# Autodesk Inventor assembly: Custom Lift
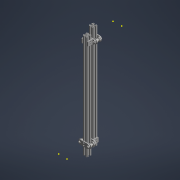
[picture p0: Inventor's stored thumbnail of the model, 180x180]
Saved by Autodesk Inventor 2022 (Build 260153000, 153)
## iProperties
Part Number: Custom Lift
Document SubType Name: Assembly
Designer: izack
Author: izack
## Documents named in this file (7)
- D:\Robotics\ComputerAidedDesign\2021-22\FTC\#12456 Big Red\Verical lift\Custom Lift\Custom Lift.iam
- D:\Robotics\ComputerAidedDesign\2021-22\FTC\#12456 Big Red\Verical lift\Custom Lift\15mm Extrusion - 420mm - 90° Ends.ipt
- D:\Robotics\ComputerAidedDesign\2021-22\FTC\#12456 Big Red\Verical lift\Custom Lift\8mm x 12mm x 3.5mm Flanged Bearing - 10 Pack.ipt
- D:\Robotics\ComputerAidedDesign\2021-22\FTC\#12456 Big Red\Verical lift\Custom Lift\Stationary Bracket.ipt
- D:\Robotics\ComputerAidedDesign\2021-22\FTC\#12456 Big Red\Verical lift\Custom Lift\5mm Hex to 8mm Round Bearing Insert - 20 Pack.ipt
- D:\Robotics\ComputerAidedDesign\2021-22\FTC\#12456 Big Red\Verical lift\Custom Lift\Stationary bracket aligner.ipt
- D:\Robotics\ComputerAidedDesign\2021-22\FTC\#12456 Big Red\Verical lift\Custom Lift\5mm x 90mm Hex Shaft - 4 Pack.ipt
## Components (26 placed, 6 different names)
1. 15mm Extrusion - 420mm - 90° Ends:1 — Mate:2, Flush:1, Tangent:1, Tangent:2, Tangent:3, Tangent:4, Tangent:5, Tangent:6, Tangent:7, Mate:16, Mate:21, Mate:22, Flush:12
2. 8mm x 12mm x 3.5mm Flanged Bearing - 10 Pack:1 — Mate:13, Mate:14, Tangent:6, Tangent:7
3. 8mm x 12mm x 3.5mm Flanged Bearing - 10 Pack:2 — Mate:12, Mate:15, Tangent:4, Tangent:5
4. 8mm x 12mm x 3.5mm Flanged Bearing - 10 Pack:3 — Mate:5, Tangent:3, Mate:8, Mate:9
5. 8mm x 12mm x 3.5mm Flanged Bearing - 10 Pack:4 — Mate:5, Tangent:1, Tangent:2, Mate:10, Mate:11
6. 15mm Extrusion - 420mm - 90° Ends:2 — Mate:2, Flush:1, Mate:6, Mate:7, Flush:11, Tangent:8, Tangent:9, Tangent:10, Tangent:11, Tangent:12, Tangent:13, Tangent:14, Tangent:15, Mate:31
7. Stationary Bracket:1 — Mate:6, Mate:7, Flush:3, Flush:6, Flush:7, Flush:8, Mate:18, Flush:11
8. 5mm Hex to 8mm Round Bearing Insert - 20 Pack:1 — Mate:10, Mate:11, Flush:4, Mate:20
9. 5mm Hex to 8mm Round Bearing Insert - 20 Pack:2 — Mate:8, Mate:9, Flush:3, Flush:4, Mate:19
10. 5mm Hex to 8mm Round Bearing Insert - 20 Pack:3 — Mate:12, Mate:15, Flush:5, Mate:17
11. 5mm Hex to 8mm Round Bearing Insert - 20 Pack:4 — Mate:13, Mate:14, Flush:5, Flush:6
12. Stationary bracket aligner:1 — Mate:16, Flush:7, Flush:8, Flush:9, Flush:10
13. 5mm x 90mm Hex Shaft - 4 Pack:1 — Mate:19, Mate:20, Flush:9
14. 5mm x 90mm Hex Shaft - 4 Pack:2 — Mate:17, Mate:18, Flush:10
15. Stationary Bracket:2 — Mate:21, Mate:22, Flush:12, Flush:15, Flush:16, Flush:17, Mate:32
16. 8mm x 12mm x 3.5mm Flanged Bearing - 10 Pack:5 — Tangent:9, Tangent:14, Mate:23, Mate:29
17. 8mm x 12mm x 3.5mm Flanged Bearing - 10 Pack:6 — Tangent:10, Tangent:15, Mate:25, Mate:28
18. 8mm x 12mm x 3.5mm Flanged Bearing - 10 Pack:7 — Tangent:11, Tangent:12, Mate:26, Mate:27
19. 8mm x 12mm x 3.5mm Flanged Bearing - 10 Pack:8 — Tangent:8, Tangent:13, Mate:24, Mate:30
20. 5mm Hex to 8mm Round Bearing Insert - 20 Pack:5 — Mate:23, Mate:29, Flush:14, Flush:15
21. 5mm Hex to 8mm Round Bearing Insert - 20 Pack:6 — Mate:24, Mate:30, Flush:13, Flush:16
22. 5mm Hex to 8mm Round Bearing Insert - 20 Pack:7 — Mate:25, Mate:28, Flush:14
23. 5mm Hex to 8mm Round Bearing Insert - 20 Pack:8 — Mate:26, Mate:27, Flush:13
24. Stationary bracket aligner:2 — Mate:31, Flush:17, Mate:32, Mate:33, Mate:34, Mate:35, Mate:36, Flush:18, Flush:19
25. 5mm x 90mm Hex Shaft - 4 Pack:3 — Mate:34, Mate:35, Flush:19
26. 5mm x 90mm Hex Shaft - 4 Pack:4 — Mate:33, Mate:36, Flush:18
## Relationships (66: Mate 33, Flush 18, Tangent 15)
- Mate:2 (4 mm): 15mm Extrusion - 420mm - 90° Ends:1 ↔ 15mm Extrusion - 420mm - 90° Ends:2
- Flush:1: 15mm Extrusion - 420mm - 90° Ends:1 ↔ 15mm Extrusion - 420mm - 90° Ends:2
- Mate:5: 8mm x 12mm x 3.5mm Flanged Bearing - 10 Pack:3 ↔ 8mm x 12mm x 3.5mm Flanged Bearing - 10 Pack:4
- Tangent:1: 15mm Extrusion - 420mm - 90° Ends:1 ↔ 8mm x 12mm x 3.5mm Flanged Bearing - 10 Pack:4
- Tangent:2: 15mm Extrusion - 420mm - 90° Ends:1 ↔ 8mm x 12mm x 3.5mm Flanged Bearing - 10 Pack:4
- Tangent:3: 15mm Extrusion - 420mm - 90° Ends:1 ↔ 8mm x 12mm x 3.5mm Flanged Bearing - 10 Pack:3
- Mate:6: 15mm Extrusion - 420mm - 90° Ends:2 ↔ Stationary Bracket:1
- Mate:7: 15mm Extrusion - 420mm - 90° Ends:2 ↔ Stationary Bracket:1
- Mate:8: 8mm x 12mm x 3.5mm Flanged Bearing - 10 Pack:3 ↔ 5mm Hex to 8mm Round Bearing Insert - 20 Pack:2
- Mate:9: 8mm x 12mm x 3.5mm Flanged Bearing - 10 Pack:3 ↔ 5mm Hex to 8mm Round Bearing Insert - 20 Pack:2
- Flush:3: Stationary Bracket:1 ↔ 5mm Hex to 8mm Round Bearing Insert - 20 Pack:2
- Mate:10: 8mm x 12mm x 3.5mm Flanged Bearing - 10 Pack:4 ↔ 5mm Hex to 8mm Round Bearing Insert - 20 Pack:1
- Mate:11: 8mm x 12mm x 3.5mm Flanged Bearing - 10 Pack:4 ↔ 5mm Hex to 8mm Round Bearing Insert - 20 Pack:1
- Flush:4: 5mm Hex to 8mm Round Bearing Insert - 20 Pack:1 ↔ 5mm Hex to 8mm Round Bearing Insert - 20 Pack:2
- Mate:12: 8mm x 12mm x 3.5mm Flanged Bearing - 10 Pack:2 ↔ 5mm Hex to 8mm Round Bearing Insert - 20 Pack:3
- Mate:13: 8mm x 12mm x 3.5mm Flanged Bearing - 10 Pack:1 ↔ 5mm Hex to 8mm Round Bearing Insert - 20 Pack:4
- Mate:14: 8mm x 12mm x 3.5mm Flanged Bearing - 10 Pack:1 ↔ 5mm Hex to 8mm Round Bearing Insert - 20 Pack:4
- Mate:15: 8mm x 12mm x 3.5mm Flanged Bearing - 10 Pack:2 ↔ 5mm Hex to 8mm Round Bearing Insert - 20 Pack:3
- Tangent:4: 15mm Extrusion - 420mm - 90° Ends:1 ↔ 8mm x 12mm x 3.5mm Flanged Bearing - 10 Pack:2
- Tangent:5: 15mm Extrusion - 420mm - 90° Ends:1 ↔ 8mm x 12mm x 3.5mm Flanged Bearing - 10 Pack:2
- Tangent:6: 15mm Extrusion - 420mm - 90° Ends:1 ↔ 8mm x 12mm x 3.5mm Flanged Bearing - 10 Pack:1
- Tangent:7: 15mm Extrusion - 420mm - 90° Ends:1 ↔ 8mm x 12mm x 3.5mm Flanged Bearing - 10 Pack:1
- Flush:5: 5mm Hex to 8mm Round Bearing Insert - 20 Pack:3 ↔ 5mm Hex to 8mm Round Bearing Insert - 20 Pack:4
- Flush:6: Stationary Bracket:1 ↔ 5mm Hex to 8mm Round Bearing Insert - 20 Pack:4
- Mate:16: 15mm Extrusion - 420mm - 90° Ends:1 ↔ Stationary bracket aligner:1
- Flush:7: Stationary Bracket:1 ↔ Stationary bracket aligner:1
- Flush:8: Stationary Bracket:1 ↔ Stationary bracket aligner:1
- Mate:17: 5mm Hex to 8mm Round Bearing Insert - 20 Pack:3 ↔ 5mm x 90mm Hex Shaft - 4 Pack:2
- Mate:18: Stationary Bracket:1 ↔ 5mm x 90mm Hex Shaft - 4 Pack:2
- Mate:19: 5mm Hex to 8mm Round Bearing Insert - 20 Pack:2 ↔ 5mm x 90mm Hex Shaft - 4 Pack:1
- Mate:20: 5mm Hex to 8mm Round Bearing Insert - 20 Pack:1 ↔ 5mm x 90mm Hex Shaft - 4 Pack:1
- Flush:9 (-2 mm): Stationary bracket aligner:1 ↔ 5mm x 90mm Hex Shaft - 4 Pack:1
- Flush:10 (-2 mm): Stationary bracket aligner:1 ↔ 5mm x 90mm Hex Shaft - 4 Pack:2
- Flush:11 (10 mm): 15mm Extrusion - 420mm - 90° Ends:2 ↔ Stationary Bracket:1
- Mate:21: 15mm Extrusion - 420mm - 90° Ends:1 ↔ Stationary Bracket:2
- Mate:22: 15mm Extrusion - 420mm - 90° Ends:1 ↔ Stationary Bracket:2
- Flush:12 (10 mm): 15mm Extrusion - 420mm - 90° Ends:1 ↔ Stationary Bracket:2
- Tangent:8: 15mm Extrusion - 420mm - 90° Ends:2 ↔ 8mm x 12mm x 3.5mm Flanged Bearing - 10 Pack:8
- Tangent:9: 15mm Extrusion - 420mm - 90° Ends:2 ↔ 8mm x 12mm x 3.5mm Flanged Bearing - 10 Pack:5
- Tangent:10: 15mm Extrusion - 420mm - 90° Ends:2 ↔ 8mm x 12mm x 3.5mm Flanged Bearing - 10 Pack:6
- Tangent:11: 15mm Extrusion - 420mm - 90° Ends:2 ↔ 8mm x 12mm x 3.5mm Flanged Bearing - 10 Pack:7
- Tangent:12: 15mm Extrusion - 420mm - 90° Ends:2 ↔ 8mm x 12mm x 3.5mm Flanged Bearing - 10 Pack:7
- Tangent:13: 15mm Extrusion - 420mm - 90° Ends:2 ↔ 8mm x 12mm x 3.5mm Flanged Bearing - 10 Pack:8
- Tangent:14: 15mm Extrusion - 420mm - 90° Ends:2 ↔ 8mm x 12mm x 3.5mm Flanged Bearing - 10 Pack:5
- Tangent:15: 15mm Extrusion - 420mm - 90° Ends:2 ↔ 8mm x 12mm x 3.5mm Flanged Bearing - 10 Pack:6
- Mate:23: 8mm x 12mm x 3.5mm Flanged Bearing - 10 Pack:5 ↔ 5mm Hex to 8mm Round Bearing Insert - 20 Pack:5
- Mate:24: 8mm x 12mm x 3.5mm Flanged Bearing - 10 Pack:8 ↔ 5mm Hex to 8mm Round Bearing Insert - 20 Pack:6
- Mate:25: 8mm x 12mm x 3.5mm Flanged Bearing - 10 Pack:6 ↔ 5mm Hex to 8mm Round Bearing Insert - 20 Pack:7
- Mate:26: 8mm x 12mm x 3.5mm Flanged Bearing - 10 Pack:7 ↔ 5mm Hex to 8mm Round Bearing Insert - 20 Pack:8
- Mate:27: 8mm x 12mm x 3.5mm Flanged Bearing - 10 Pack:7 ↔ 5mm Hex to 8mm Round Bearing Insert - 20 Pack:8
- Mate:28: 8mm x 12mm x 3.5mm Flanged Bearing - 10 Pack:6 ↔ 5mm Hex to 8mm Round Bearing Insert - 20 Pack:7
- Mate:29: 8mm x 12mm x 3.5mm Flanged Bearing - 10 Pack:5 ↔ 5mm Hex to 8mm Round Bearing Insert - 20 Pack:5
- Mate:30: 8mm x 12mm x 3.5mm Flanged Bearing - 10 Pack:8 ↔ 5mm Hex to 8mm Round Bearing Insert - 20 Pack:6
- Flush:13: 5mm Hex to 8mm Round Bearing Insert - 20 Pack:6 ↔ 5mm Hex to 8mm Round Bearing Insert - 20 Pack:8
- Flush:14: 5mm Hex to 8mm Round Bearing Insert - 20 Pack:5 ↔ 5mm Hex to 8mm Round Bearing Insert - 20 Pack:7
- Flush:15: Stationary Bracket:2 ↔ 5mm Hex to 8mm Round Bearing Insert - 20 Pack:5
- Flush:16: Stationary Bracket:2 ↔ 5mm Hex to 8mm Round Bearing Insert - 20 Pack:6
- Mate:31: 15mm Extrusion - 420mm - 90° Ends:2 ↔ Stationary bracket aligner:2
- Flush:17: Stationary Bracket:2 ↔ Stationary bracket aligner:2
- Mate:32: Stationary Bracket:2 ↔ Stationary bracket aligner:2
- Mate:33: Stationary bracket aligner:2 ↔ 5mm x 90mm Hex Shaft - 4 Pack:4
- Mate:34: Stationary bracket aligner:2 ↔ 5mm x 90mm Hex Shaft - 4 Pack:3
- Mate:35: Stationary bracket aligner:2 ↔ 5mm x 90mm Hex Shaft - 4 Pack:3
- Mate:36: Stationary bracket aligner:2 ↔ 5mm x 90mm Hex Shaft - 4 Pack:4
- Flush:18 (-2 mm): Stationary bracket aligner:2 ↔ 5mm x 90mm Hex Shaft - 4 Pack:4
- Flush:19 (-2 mm): Stationary bracket aligner:2 ↔ 5mm x 90mm Hex Shaft - 4 Pack:3
